# Autodesk Inventor assembly: anschluss_daten
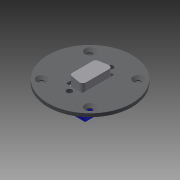
[picture p0: Inventor's stored thumbnail of the model, 180x180]
Saved by Autodesk Inventor 2016 SP2 (Build 200236200, 236)
## iProperties
Created: 2018-04-03
Part Number: anschluss_daten
Document SubType Name: Assembly
Designer: wepet
Mass: 7.17984 g
Surface Area: 59.51 cm^2
Volume: 7.17984 cm^3
Density: 1 g/cm^3
Author: wepet
## Documents named in this file (3)
- L:\Granz\RoboSAX\anschluss_daten.iam
- L:\Granz\RoboSAX\anschluss_daten_1.ipt
- L:\Granz\RoboSAX\anschluss_daten_2.ipt
## Components (2 placed, 2 different names)
1. anschluss_daten_1:1 — Drehbar:1, Drehbar:2
2. anschluss_daten_2:1 — Drehbar:1, Drehbar:2, Passend:2, Fluchtend:1
## Relationships (4: RevoluteJoint 2, Mate 1, Flush 1)
- Drehbar:1 [RevoluteJoint] (3 mm): anschluss_daten_1:1 ↔ anschluss_daten_2:1
- Drehbar:2 [RevoluteJoint] (3 mm): anschluss_daten_1:1 ↔ anschluss_daten_2:1
- Passend:2 [Mate] (-4.18 mm): anschluss_daten_2:1
- Fluchtend:1 [Flush] (-15.405 mm): anschluss_daten_2:1
